# Autodesk Inventor assembly: BaseFrame
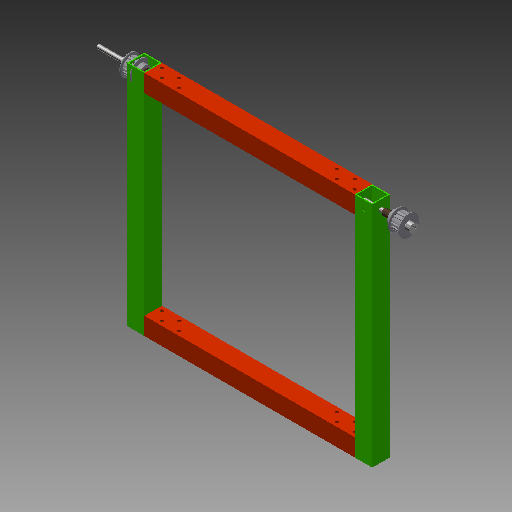
[picture p0: Inventor's stored thumbnail of the model, 512x512]
Saved by Autodesk Inventor 2019 (Build 230136000, 136)
## iProperties
Created: 2019-01-10
Part Number: BaseFrame
Document SubType Name: Assembly
Designer: james
Mass: 718.374 g
Surface Area: 2695.29 cm^2
Volume: 222.03 cm^3
Density: 3.23548 g/cm^3
Author: james
## Documents named in this file (4)
- F:\JimsDesign\2019CHS4089\BaseFrame.iam
- F:\JimsDesign\2019CHS4089\ElvCrossBeam.ipt
- F:\JimsDesign\2019CHS4089\ElvEndEffectBeam.ipt
- F:\JimsDesign\2019CHS4089\ElvShaft.iam
## Components (5 placed, 3 different names)
1. ElvCrossBeam:1 — Mate:2, Flush:3, Flush:4
2. ElvCrossBeam:2 — Mate:1, Flush:1, Flush:2, Mate:3, Flush:5, Flush:6
3. ElvEndEffectBeam:1 — Mate:1, Flush:1, Flush:2, Mate:2, Flush:3, Flush:4, Mate:4
4. ElvEndEffectBeam:2 — Mate:3, Flush:5, Flush:6
5. ElvShaft:1 [sub-assembly] — Mate:4
## Relationships (10: Flush 6, Mate 4)
- Mate:1: ElvCrossBeam:2 ↔ ElvEndEffectBeam:1
- Flush:1: ElvCrossBeam:2 ↔ ElvEndEffectBeam:1
- Flush:2: ElvCrossBeam:2 ↔ ElvEndEffectBeam:1
- Mate:2: ElvCrossBeam:1 ↔ ElvEndEffectBeam:1
- Flush:3: ElvCrossBeam:1 ↔ ElvEndEffectBeam:1
- Flush:4: ElvCrossBeam:1 ↔ ElvEndEffectBeam:1
- Mate:3: ElvCrossBeam:2 ↔ ElvEndEffectBeam:2
- Flush:5: ElvCrossBeam:2 ↔ ElvEndEffectBeam:2
- Flush:6: ElvCrossBeam:2 ↔ ElvEndEffectBeam:2
- Mate:4: ElvEndEffectBeam:1 ↔ ElvShaft:1
